# Autodesk Inventor assembly: TestRig
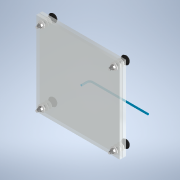
[picture p0: Inventor's stored thumbnail of the model, 180x180]
Saved by Autodesk Inventor 2020.3 (Build 243373000, 373)
## iProperties
Created: 2020-10-30
Part Number: TestRig
Document SubType Name: Assembly
Designer: Naude Conradie
Author: Naude Conradie
## Documents named in this file (8)
- C:\Users\Naude Conradie\Desktop\Repository\Masters-Project\Models\Inventor\Testing Rig\TestRig.iam
- C:\Users\Naude Conradie\Desktop\Repository\Masters-Project\Models\Inventor\Testing Rig\Plate.ipt
- C:\Users\Naude Conradie\Desktop\Repository\Masters-Project\Models\Inventor\Testing Rig\PlateHoled.ipt
- C:\Users\Naude Conradie\Desktop\Repository\Masters-Project\Models\Inventor\Testing Rig\Leg.ipt
- C:\Users\Naude Conradie\Desktop\Repository\Masters-Project\Models\Inventor\Testing Rig\Washer.ipt
- C:\Users\Naude Conradie\Desktop\Repository\Masters-Project\Models\Inventor\Testing Rig\Foot.ipt
- C:\Users\Naude Conradie\Documents\Inventor\Content Center Files\R2020\en-US\ANSI B 18.2.4.1 M(1)\ANSI B 18.2.4.1 M - M8 x 1,25Style 1.ipt
- C:\Users\Naude Conradie\Desktop\Repository\Masters-Project\Models\Inventor\Testing Rig\Pipe.ipt
## Components (27 placed, 7 different names)
1. Plate:1 — Mate:4, Flush:3, Mate:22, Mate:23, Mate:24, Mate:25, Mate:26, Mate:27, Mate:28, Mate:29, Mate:51, Mate:52, Mate:53, Mate:54, Mate:55, Mate:56, Mate:57, Mate:58, Mate:63, Mate:64, Mate:65, Mate:66
2. PlateHoled:1 — Mate:4, Flush:3, Mate:30, Mate:43, Mate:44, Mate:45, Mate:46, Mate:47, Mate:48, Mate:49, Mate:50, Flush:8, Mate:67
3. Washer:1 — Mate:22, Mate:27
4. Washer:2 — Mate:23, Mate:28
5. Washer:3 — Mate:25, Mate:29, Mate:30
6. Washer:4 — Mate:24, Mate:26
7. Foot:1 — Mate:32, Mate:35, Mate:36, Mate:50
8. Foot:2 — Mate:34, Mate:39, Mate:41, Mate:48
9. Foot:3 — Mate:31, Mate:37, Mate:38, Mate:49
10. Foot:4 — Mate:33, Mate:40, Mate:42, Mate:47
11. Leg:1 — Mate:31, Flush:4
12. Leg:2 — Mate:32, Flush:7
13. Leg:3 — Mate:34, Flush:5
14. Leg:4 — Mate:33, Flush:6
15. Washer:5 — Mate:37, Mate:38, Mate:45
16. Washer:6 — Mate:35, Mate:36, Mate:46
17. Washer:7 — Mate:39, Mate:41, Mate:44
18. Washer:8 — Mate:54, Mate:55, Mate:62
19. Washer:9 — Mate:53, Mate:57, Mate:59
20. Washer:10 — Mate:40, Mate:42, Mate:43
21. Washer:11 — Mate:51, Mate:56, Mate:60
22. Washer:12 — Mate:52, Mate:58, Mate:61
23. Hex Nut Metric M8 x 1,25:1 — Mate:59, Mate:66, Flush:4
24. Hex Nut Metric M8 x 1,25:2 — Mate:60, Mate:65, Flush:7
25. Hex Nut Metric M8 x 1,25:3 — Mate:61, Mate:63, Flush:5
26. Hex Nut Metric M8 x 1,25:4 — Mate:62, Mate:64, Flush:6
27. Pipe:1 — Flush:8, Mate:67
## Relationships (53: Mate 47, Flush 6)
- Mate:4: Plate:1 ↔ PlateHoled:1
- Flush:3: Plate:1 ↔ PlateHoled:1
- Mate:22: Plate:1 ↔ Washer:1
- Mate:23: Plate:1 ↔ Washer:2
- Mate:24: Plate:1 ↔ Washer:4
- Mate:25: Plate:1 ↔ Washer:3
- Mate:26: Plate:1 ↔ Washer:4
- Mate:27: Plate:1 ↔ Washer:1
- Mate:28: Plate:1 ↔ Washer:2
- Mate:29: Plate:1 ↔ Washer:3
- Mate:30: PlateHoled:1 ↔ Washer:3
- Mate:31: Foot:3 ↔ Leg:1
- Mate:32: Foot:1 ↔ Leg:2
- Mate:33: Foot:4 ↔ Leg:4
- Mate:34: Foot:2 ↔ Leg:3
- Mate:35: Foot:1 ↔ Washer:6
- Mate:36: Foot:1 ↔ Washer:6
- Mate:37: Foot:3 ↔ Washer:5
- Mate:38: Foot:3 ↔ Washer:5
- Mate:39: Foot:2 ↔ Washer:7
- Mate:40: Foot:4 ↔ Washer:10
- Mate:41: Foot:2 ↔ Washer:7
- Mate:42: Foot:4 ↔ Washer:10
- Mate:43: PlateHoled:1 ↔ Washer:10
- Mate:44: PlateHoled:1 ↔ Washer:7
- Mate:45: PlateHoled:1 ↔ Washer:5
- Mate:46: PlateHoled:1 ↔ Washer:6
- Mate:47: PlateHoled:1 ↔ Foot:4
- Mate:48: PlateHoled:1 ↔ Foot:2
- Mate:49: PlateHoled:1 ↔ Foot:3
- Mate:50: PlateHoled:1 ↔ Foot:1
- Mate:51: Plate:1 ↔ Washer:11
- Mate:52: Plate:1 ↔ Washer:12
- Mate:53: Plate:1 ↔ Washer:9
- Mate:54: Plate:1 ↔ Washer:8
- Mate:55: Plate:1 ↔ Washer:8
- Mate:56: Plate:1 ↔ Washer:11
- Mate:57: Plate:1 ↔ Washer:9
- Mate:58: Plate:1 ↔ Washer:12
- Mate:59: Washer:9 ↔ Hex Nut Metric M8 x 1,25:1
- Mate:60: Washer:11 ↔ Hex Nut Metric M8 x 1,25:2
- Mate:61: Washer:12 ↔ Hex Nut Metric M8 x 1,25:3
- Mate:62: Washer:8 ↔ Hex Nut Metric M8 x 1,25:4
- Mate:63: Plate:1 ↔ Hex Nut Metric M8 x 1,25:3
- Mate:64: Plate:1 ↔ Hex Nut Metric M8 x 1,25:4
- Mate:65: Plate:1 ↔ Hex Nut Metric M8 x 1,25:2
- Mate:66: Plate:1 ↔ Hex Nut Metric M8 x 1,25:1
- Flush:4 (-10 mm): Leg:1 ↔ Hex Nut Metric M8 x 1,25:1
- Flush:5 (-10 mm): Leg:3 ↔ Hex Nut Metric M8 x 1,25:3
- Flush:6 (-10 mm): Leg:4 ↔ Hex Nut Metric M8 x 1,25:4
- Flush:7 (-10 mm): Leg:2 ↔ Hex Nut Metric M8 x 1,25:2
- Flush:8: PlateHoled:1 ↔ Pipe:1
- Mate:67: PlateHoled:1 ↔ Pipe:1
